# Autodesk Inventor assembly: Bearingw-screws
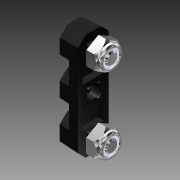
[picture p0: Inventor's stored thumbnail of the model, 180x180]
Saved by Autodesk Inventor 2014 (Build 180170000, 170)
## iProperties
Created: 2014-08-19
Part Number: Bearingw-screws
Document SubType Name: Assembly
Designer: Josef
Author: Josef
## Documents named in this file (4)
- C:\Users\Josef\Documents\Vex parts\Bearingw-screws.iam
- C:\Users\Josef\Documents\Vex parts\Other Parts\Bearing Flat, Delrin.ipt
- C:\Users\Josef\Documents\Vex parts\Screws & Nuts\Screw 8-32 x 0.500''-Silver.ipt
- C:\Users\Josef\Documents\Vex parts\Screws & Nuts\Nut 8-32 Nylock.ipt
## Components (5 placed, 3 different names)
1. Bearing Flat, Delrin:1 — Insert:1, Insert:2
2. Screw 8-32 x 0.500''-Silver:1 — Insert:1, Mate:4
3. Screw 8-32 x 0.500''-Silver:2 — Insert:2, Mate:5
4. Nut 8-32 Nylock:1 — Mate:5
5. Nut 8-32 Nylock:2 — Mate:4
## Relationships (4: Insert 2, Mate 2)
- Insert:1: Bearing Flat, Delrin:1 ↔ Screw 8-32 x 0.500''-Silver:1
- Insert:2: Bearing Flat, Delrin:1 ↔ Screw 8-32 x 0.500''-Silver:2
- Mate:4: Screw 8-32 x 0.500''-Silver:1 ↔ Nut 8-32 Nylock:2
- Mate:5: Screw 8-32 x 0.500''-Silver:2 ↔ Nut 8-32 Nylock:1
